# Autodesk Inventor assembly: Input Potentiometer
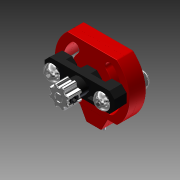
[picture p0: Inventor's stored thumbnail of the model, 180x180]
Saved by Autodesk Inventor 2012 (Build 160160000, 160)
## iProperties
Created: 2011-09-15
Part Number: Input Potentiometer
Document SubType Name: Assembly
Designer: Wade
Author: Wade
## Documents named in this file (9)
- C:\Users\Wade\Documents\1103 Robot - CAD Assembly\Input Potentiometer.iam
- C:\Users\Wade\Documents\24C VEX CAD Files\Motors & Sensors\Potentiometer.iam
- C:\Users\Wade\Documents\24C VEX CAD Files\Other Parts\Bearing Flat, Delrin.ipt
- C:\Users\Wade\Documents\24C VEX CAD Files\Other Parts\Shaft Collar (Custom).ipt
- C:\Users\Wade\Documents\24C VEX CAD Files\Other Parts\Shaft Collar (with Set Screw Installed).ipt
- C:\Users\Wade\Documents\24C VEX CAD Files\Screws & Nuts\Screw 8-32 x 0.875''-Silver.ipt
- C:\Users\Wade\Documents\24C VEX CAD Files\Screws & Nuts\Nut 8-32 Nylock.ipt
- C:\Users\Wade\Documents\24C VEX CAD Files\Washers & Spacers\Spacer (Thin), 4.6mm.ipt
- C:\Users\Wade\Documents\24C VEX CAD Files\Drive Shafts\Drive Shaft (Square Bar) 1.25''.ipt
## Components (10 placed, 8 different names)
1. Potentiometer:1 [sub-assembly] — Mate:1, Mate:2, Flush:1, Mate:3, Mate:4, Mate:5, Mate:6, Mate:12, Mate:14
2. Drive Shaft (Square Bar) 1.25'':1 — Mate:1, Mate:2, Flush:1, Angle:1, Flush:2, Angle:2
3. Bearing Flat, Delrin:1 — Mate:5, Mate:6, Mate:7, Mate:8, Mate:9, Mate:10, Mate:15, Mate:16
4. Shaft Collar (Custom):1 — Mate:16, Mate:17, Flush:2, Angle:2
5. Shaft Collar (with Set Screw Installed):1 — Mate:3, Mate:4, Angle:1
6. Screw 8-32 x 0.875''-Silver:1 — Mate:7, Mate:10, Mate:11
7. Screw 8-32 x 0.875''-Silver:2 — Mate:8, Mate:9, Mate:13
8. Nut 8-32 Nylock:1 — Mate:13, Mate:14
9. Nut 8-32 Nylock:2 — Mate:11, Mate:12
10. Spacer (Thin), 4.6mm:1 — Mate:15, Mate:17
## Relationships (21: Mate 17, Flush 2, Angle 2)
- Mate:1 (-0.3937 mm): Potentiometer:1 ↔ Drive Shaft (Square Bar) 1.25'':1
- Mate:2 (-1.5875 mm): Potentiometer:1 ↔ Drive Shaft (Square Bar) 1.25'':1
- Flush:1 (-17.0434 mm): Potentiometer:1 ↔ Drive Shaft (Square Bar) 1.25'':1
- Mate:3: Potentiometer:1 ↔ Shaft Collar (with Set Screw Installed):1
- Mate:4: Potentiometer:1 ↔ Shaft Collar (with Set Screw Installed):1
- Angle:1 (0 deg): Drive Shaft (Square Bar) 1.25'':1 ↔ Shaft Collar (with Set Screw Installed):1
- Mate:5: Potentiometer:1 ↔ Bearing Flat, Delrin:1
- Mate:6: Potentiometer:1 ↔ Bearing Flat, Delrin:1
- Mate:7: Bearing Flat, Delrin:1 ↔ Screw 8-32 x 0.875''-Silver:1
- Mate:8: Bearing Flat, Delrin:1 ↔ Screw 8-32 x 0.875''-Silver:2
- Mate:9 (1.1684 mm): Bearing Flat, Delrin:1 ↔ Screw 8-32 x 0.875''-Silver:2
- Mate:10 (1.1684 mm): Bearing Flat, Delrin:1 ↔ Screw 8-32 x 0.875''-Silver:1
- Mate:11: Screw 8-32 x 0.875''-Silver:1 ↔ Nut 8-32 Nylock:2
- Mate:12: Potentiometer:1 ↔ Nut 8-32 Nylock:2
- Mate:13: Screw 8-32 x 0.875''-Silver:2 ↔ Nut 8-32 Nylock:1
- Mate:14: Potentiometer:1 ↔ Nut 8-32 Nylock:1
- Mate:15: Bearing Flat, Delrin:1 ↔ Spacer (Thin), 4.6mm:1
- Mate:16: Bearing Flat, Delrin:1 ↔ Shaft Collar (Custom):1
- Mate:17: Shaft Collar (Custom):1 ↔ Spacer (Thin), 4.6mm:1
- Flush:2: Drive Shaft (Square Bar) 1.25'':1 ↔ Shaft Collar (Custom):1
- Angle:2 (0 deg): Drive Shaft (Square Bar) 1.25'':1 ↔ Shaft Collar (Custom):1
